# Autodesk Inventor assembly: Montagem1
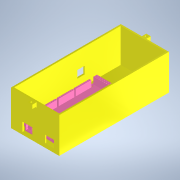
[picture p0: Inventor's stored thumbnail of the model, 180x180]
Saved by Autodesk Inventor 2022 (Build 260153000, 153)
## iProperties
Created: 2024-03-03
Part Number: Montagem1
Document SubType Name: Assembly
Designer: Daniel
Author: Daniel
## Documents named in this file (3)
- C:\Users\Daniel\Documents\Inventor\prototipoV4\Montagem1.iam
- C:\Users\Daniel\Documents\Inventor\prototipoV4\ArduinoMega_STEP_AP203.ipt
- C:\Users\Daniel\Documents\Inventor\prototipoV4\basecaixa.ipt
## Components (2 placed, 2 different names)
1. ArduinoMega_STEP_AP203:1 — Coincidente:1
2. basecaixa:1 — Coincidente:1
## Relationships (1: Mate 1)
- Coincidente:1 [Mate]: ArduinoMega_STEP_AP203:1 ↔ basecaixa:1
